# Autodesk Inventor assembly: Race Inner
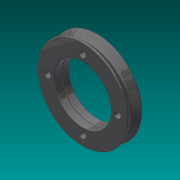
[picture p0: Inventor's stored thumbnail of the model, 180x180]
Saved by Autodesk Inventor 2020.2 (Build 242310000, 310)
## iProperties
Created: 2020-05-22
Part Number: Race Inner
Document SubType Name: Assembly
Designer: Administrator
Title: Race Inner
Author: Administrator
## Documents named in this file (3)
- C:\Users\Svend\OneDrive\Documents\GitHub\BeerMinder\3D-model\bearings\slewbearing\Race Inner.iam
- C:\Users\Svend\OneDrive\Documents\GitHub\BeerMinder\3D-model\bearings\slewbearing\Race Inner Bottom.ipt
- C:\Users\Svend\OneDrive\Documents\GitHub\BeerMinder\3D-model\bearings\slewbearing\Race Inner Top.ipt
## Components (2 placed, 2 different names)
1. Race Inner Bottom:1 — Mate:1, Mate:2, Mate:3
2. Race Inner Top:1 — Mate:1, Mate:2, Mate:3
## Relationships (3: Mate 3)
- Mate:1: Race Inner Bottom:1 ↔ Race Inner Top:1
- Mate:2: Race Inner Bottom:1 ↔ Race Inner Top:1
- Mate:3: Race Inner Bottom:1 ↔ Race Inner Top:1
